# Autodesk Inventor assembly: DriveTrainBase
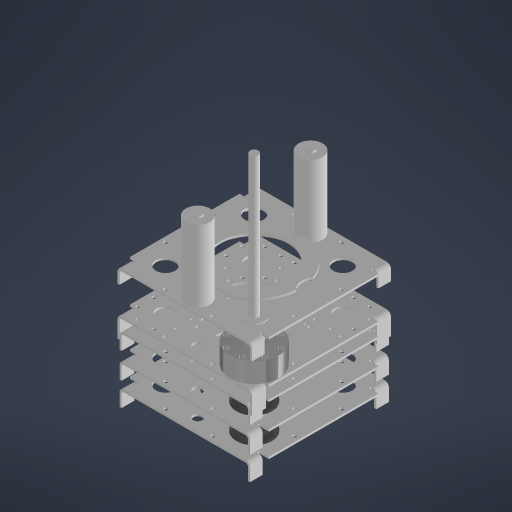
[picture p0: Inventor's stored thumbnail of the model, 512x512]
Saved by Autodesk Inventor 2024 (Build 280153000, 153)
## iProperties
Created: 2025-02-12
Part Number: DriveTrainBase
Document SubType Name: Assembly
Designer: Tommy Rohmann
Author: Tommy Rohmann
## Documents named in this file (9)
- C:\Users\Tommy Rohmann\OneDrive\Projects\Microgravity-Press-Washing-Machine\System Design and Documentation\Inventor Design Project\SUBDriveTrainBase.iam
- C:\Users\Tommy Rohmann\OneDrive\Projects\Microgravity-Press-Washing-Machine\System Design and Documentation\Inventor Design Project\LoadCellBase.ipt
- C:\Users\Tommy Rohmann\OneDrive\Projects\Microgravity-Press-Washing-Machine\System Design and Documentation\Inventor Design Project\LoadCell.ipt
- C:\Users\Tommy Rohmann\OneDrive\Projects\Microgravity-Press-Washing-Machine\System Design and Documentation\Inventor Design Project\DriveMotor.ipt
- C:\Users\Tommy Rohmann\OneDrive\Projects\Microgravity-Press-Washing-Machine\System Design and Documentation\Inventor Design Project\SUBDriveShaftACME.iam
- C:\Users\Tommy Rohmann\OneDrive\Projects\Microgravity-Press-Washing-Machine\System Design and Documentation\Inventor Design Project\TopBase.ipt
- C:\Users\Tommy Rohmann\OneDrive\Projects\Microgravity-Press-Washing-Machine\System Design and Documentation\Inventor Design Project\LAYOUT.ipt
- C:\Users\Tommy Rohmann\OneDrive\Projects\Microgravity-Press-Washing-Machine\System Design and Documentation\Inventor Design Project\ChainBase.ipt
- C:\Users\Tommy Rohmann\OneDrive\Projects\Microgravity-Press-Washing-Machine\System Design and Documentation\Inventor Design Project\WashChamberRetainerRing.ipt
## Components (11 placed, 8 different names)
1. LoadCellBase:1 — Mate:22, Flush:1, Mate:59, Mate:61, Mate:62
2. DriveMotor:1 — Mate:20, Mate:21
3. SUBDriveShaftACME:1 [sub-assembly] — Mate:15, Mate:16, Mate:49, Mate:50, Mate:51, Mate:53, Mate:54, Mate:55, Flush:1, Mate:59, Mate:60
4. LAYOUT:1
5. TopBase:1 — Mate:15, Mate:16, Mate:18, Mate:19, Mate:20, Mate:21, Mate:22, Mate:47, Mate:48, Mate:52, Mate:56, Mate:57, Mate:58
6. DriveMotor:3 — Mate:18, Mate:19
7. ChainBase:1 — Mate:47, Mate:50, Mate:55
8. ChainBase:2 — Mate:48, Mate:49, Mate:51
9. ChainBase:3 — Mate:52, Mate:53, Mate:54
10. WashChamberRetainerRing:1 — Mate:56, Mate:57, Mate:58
11. LoadCell:1 — Mate:60, Mate:61, Mate:62
## Relationships (24: Mate 23, Flush 1)
- Mate:15: SUBDriveShaftACME:1 ↔ TopBase:1
- Mate:16: SUBDriveShaftACME:1 ↔ TopBase:1
- Mate:18: TopBase:1 ↔ DriveMotor:3
- Mate:19: TopBase:1 ↔ DriveMotor:3
- Mate:20: DriveMotor:1 ↔ TopBase:1
- Mate:21: DriveMotor:1 ↔ TopBase:1
- Mate:22: LoadCellBase:1 ↔ TopBase:1
- Mate:47: TopBase:1 ↔ ChainBase:1
- Mate:48: TopBase:1 ↔ ChainBase:2
- Mate:49: SUBDriveShaftACME:1 ↔ ChainBase:2
- Mate:50: SUBDriveShaftACME:1 ↔ ChainBase:1
- Mate:51: SUBDriveShaftACME:1 ↔ ChainBase:2
- Mate:52: TopBase:1 ↔ ChainBase:3
- Mate:53: SUBDriveShaftACME:1 ↔ ChainBase:3
- Mate:54: SUBDriveShaftACME:1 ↔ ChainBase:3
- Mate:55: SUBDriveShaftACME:1 ↔ ChainBase:1
- Mate:56: TopBase:1 ↔ WashChamberRetainerRing:1
- Mate:57: TopBase:1 ↔ WashChamberRetainerRing:1
- Mate:58 (3.175 mm): TopBase:1 ↔ WashChamberRetainerRing:1
- Flush:1: LoadCellBase:1 ↔ SUBDriveShaftACME:1
- Mate:59: LoadCellBase:1 ↔ SUBDriveShaftACME:1
- Mate:60: SUBDriveShaftACME:1 ↔ LoadCell:1
- Mate:61: LoadCellBase:1 ↔ LoadCell:1
- Mate:62: LoadCellBase:1 ↔ LoadCell:1
